# Autodesk Inventor assembly: Bended Counter
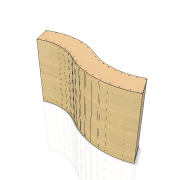
[picture p0: Inventor's stored thumbnail of the model, 180x180]
Saved by Autodesk Inventor 2024 (Build 280153000, 153)
## iProperties
RuleStatus: InUse
Created: 2019-11-14
Part Number: Bended Counter
Document SubType Name: Assembly
Designer: SauliusD
Author: SauliusD
## Documents named in this file (9)
- C:\W4INV 2024 Design\PROJECTS\Samples\Bended counter\Bended Counter.iam
- C:\W4INV 2024 Design\PROJECTS\Samples\Bended counter\Bottom.ipt
- C:\W4INV 2024 Design\PROJECTS\Samples\Bended counter\Strut.ipt
- C:\W4INV 2024 Design\PROJECTS\Samples\Bended counter\Top.ipt
- C:\W4INV 2024 Design\_LIBRARY\Fixed joints\Confirmat\CONFIRMAT\Confirmat L50 & Cap D10 NB T18 PB T 18.ipt
- C:\W4INV 2024 Design\PROJECTS\Samples\Bended counter\Bended Counter.ipt
- C:\W4INV 2024 Design\_LIBRARY\Fixed joints\Confirmat\CONFIRMAT\Confirmat L50 NB T18 PB T 18.ipt
- C:\W4INV 2024 Design\PROJECTS\Samples\Bended counter\Side Cover_1.ipt
- C:\W4INV 2024 Design\LIBRARY\Fixed joints\Confirmat\CONFIRMAT.ipt
## Components (84 placed, 7 different names)
1. Skeleton
2. Bottom:1 — Insert:3, Insert:4
3. Top:1 — Insert:1, Insert:2
4. Side Cover_1:1
5. Confirmat L50 & Cap D10 NB T18 PB T 18:1 — Insert:1
6. Confirmat L50 & Cap D10 NB T18 PB T 18:2 — Insert:2
7. Confirmat L50 & Cap D10 NB T18 PB T 18:3
8. Confirmat L50 & Cap D10 NB T18 PB T 18:4
9. Confirmat L50 & Cap D10 NB T18 PB T 18:5
10. Confirmat L50 & Cap D10 NB T18 PB T 18:6
11. Confirmat L50 & Cap D10 NB T18 PB T 18:7
12. Confirmat L50 & Cap D10 NB T18 PB T 18:8
13. Confirmat L50 & Cap D10 NB T18 PB T 18:9
14. Confirmat L50 & Cap D10 NB T18 PB T 18:10
15. Confirmat L50 & Cap D10 NB T18 PB T 18:11
16. Confirmat L50 & Cap D10 NB T18 PB T 18:12
17. Confirmat L50 & Cap D10 NB T18 PB T 18:13
18. Confirmat L50 & Cap D10 NB T18 PB T 18:14
19. Confirmat L50 & Cap D10 NB T18 PB T 18:15
20. Confirmat L50 & Cap D10 NB T18 PB T 18:16
21. Confirmat L50 & Cap D10 NB T18 PB T 18:17
22. Confirmat L50 & Cap D10 NB T18 PB T 18:18
23. Confirmat L50 & Cap D10 NB T18 PB T 18:19
24. Confirmat L50 & Cap D10 NB T18 PB T 18:20
25. Confirmat L50 & Cap D10 NB T18 PB T 18:21
26. Confirmat L50 & Cap D10 NB T18 PB T 18:22
27. Confirmat L50 & Cap D10 NB T18 PB T 18:23
28. Confirmat L50 & Cap D10 NB T18 PB T 18:24
29. Confirmat L50 & Cap D10 NB T18 PB T 18:25
30. Confirmat L50 & Cap D10 NB T18 PB T 18:26
31. Confirmat L50 & Cap D10 NB T18 PB T 18:27
32. Confirmat L50 & Cap D10 NB T18 PB T 18:28
33. Confirmat L50 & Cap D10 NB T18 PB T 18:29
34. Confirmat L50 & Cap D10 NB T18 PB T 18:30
35. Confirmat L50 & Cap D10 NB T18 PB T 18:31
36. Confirmat L50 & Cap D10 NB T18 PB T 18:32
37. Strut:1
38. Strut:2
39. Strut:3
40. Strut:4
41. Strut:5
42. Strut:6
43. Strut:7
44. Strut:8
45. Strut:9
46. Strut:10
47. Strut:11
48. Strut:12
49. Strut:13
50. Strut:14
51. Strut:15
52. Strut:16
53. Confirmat L50 NB T18 PB T 18:33 — Insert:3
54. Confirmat L50 NB T18 PB T 18:34 — Insert:4
55. Confirmat L50 NB T18 PB T 18:35
56. Confirmat L50 NB T18 PB T 18:36
57. Confirmat L50 NB T18 PB T 18:37
58. Confirmat L50 NB T18 PB T 18:38
59. Confirmat L50 NB T18 PB T 18:39
60. Confirmat L50 NB T18 PB T 18:40
61. Confirmat L50 NB T18 PB T 18:41
62. Confirmat L50 NB T18 PB T 18:42
63. Confirmat L50 NB T18 PB T 18:43
64. Confirmat L50 NB T18 PB T 18:44
65. Confirmat L50 NB T18 PB T 18:45
66. Confirmat L50 NB T18 PB T 18:46
67. Confirmat L50 NB T18 PB T 18:47
68. Confirmat L50 NB T18 PB T 18:48
69. Confirmat L50 NB T18 PB T 18:49
70. Confirmat L50 NB T18 PB T 18:50
71. Confirmat L50 NB T18 PB T 18:51
72. Confirmat L50 NB T18 PB T 18:52
73. Confirmat L50 NB T18 PB T 18:53
74. Confirmat L50 NB T18 PB T 18:54
75. Confirmat L50 NB T18 PB T 18:55
76. Confirmat L50 NB T18 PB T 18:56
77. Confirmat L50 NB T18 PB T 18:57
78. Confirmat L50 NB T18 PB T 18:58
79. Confirmat L50 NB T18 PB T 18:59
80. Confirmat L50 NB T18 PB T 18:60
81. Confirmat L50 NB T18 PB T 18:61
82. Confirmat L50 NB T18 PB T 18:62
83. Confirmat L50 NB T18 PB T 18:63
84. Confirmat L50 NB T18 PB T 18:64
## Component patterns: (16 elements, first: Confirmat L50 & Cap D10 NB T18 PB T 18:1 + Confirmat L50 & Cap D10 NB T18 PB T 18:2), (16 elements, first: Strut:1), (16 elements, first: Confirmat L50 NB T18 PB T 18:33 + Confirmat L50 NB T18 PB T 18:34)
## Relationships (4: Insert 4)
- Insert:1: Top:1 ↔ Confirmat L50 & Cap D10 NB T18 PB T 18:1
- Insert:2: Top:1 ↔ Confirmat L50 & Cap D10 NB T18 PB T 18:2
- Insert:3: Bottom:1 ↔ Confirmat L50 NB T18 PB T 18:33
- Insert:4: Bottom:1 ↔ Confirmat L50 NB T18 PB T 18:34
